# Autodesk Inventor assembly: GP6-100
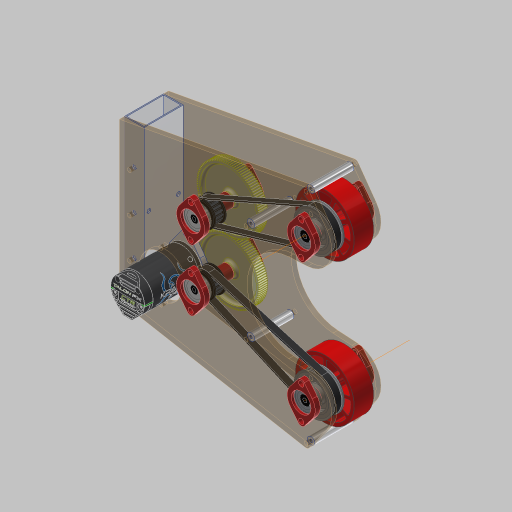
[picture p0: Inventor's stored thumbnail of the model, 512x512]
Saved by Autodesk Inventor 2023.5 (Build 275446000, 446)
## iProperties
Created: 2025-02-23
Part Number: GP6-100
Document SubType Name: Assembly
Designer: slick
Author: slick
## Documents named in this file (23)
- C:\Users\slick\OneDrive\Desktop\2025-ReefScape---CAD\Gripper\GP6\GP6-100.iam
- C:\Users\slick\OneDrive\Desktop\2025-ReefScape---CAD\Gripper\GP6\GP6-001.ipt
- C:\Users\slick\OneDrive\Desktop\2025-ReefScape---CAD\Gripper\GP6\GP6-003.ipt
- C:\Users\slick\OneDrive\Desktop\2025-ReefScape---CAD\Gripper\GP6\GP6-002.ipt
- C:\Users\slick\OneDrive\Desktop\2025-ReefScape---CAD\COMMON PARTS\BEARINGS\0_500_ID_x_1_125_OD_x_0_313_WD_Flanged_Bearing_217-2731.ipt
- C:\Users\slick\OneDrive\Desktop\2025-ReefScape---CAD\COMMON PARTS\BEARINGS\Bearing Retainer\Retainer.ipt
- C:\Users\slick\OneDrive\Desktop\2025-ReefScape---CAD\COMMON PARTS\BEARINGS\0_375_ID_x_1_125_OD_x_0_313_WD_Flanged_Bearing_217-2732.ipt
- C:\Users\slick\OneDrive\Desktop\2025-ReefScape---CAD\Gripper\GP6\GP6-005.ipt
- C:\Users\slick\OneDrive\Desktop\2025-ReefScape---CAD\Gripper\GP6\GP6-006.ipt
- C:\Users\slick\OneDrive\Desktop\2025-ReefScape---CAD\COMMON PARTS\GEARS\15t Spur Gear\15t Spur Gear.ipt
- C:\Users\slick\OneDrive\Desktop\2025-ReefScape---CAD\COMMON PARTS\GEARS\32 dp gear\100t_Aluminum_Spur_Gear_32_DP_3_8_Hex_Bore_217-5865.ipt
- C:\Users\slick\OneDrive\Desktop\2025-ReefScape---CAD\Gripper\GP6\GP6-007.ipt
- C:\Users\slick\OneDrive\Desktop\2025-ReefScape---CAD\COMMON PARTS\PULLEYS\htd\30t_x_9mm_Wide_Double_Flange_Aluminum_Pulley_HTD_5mm_1_2_Hex_Bore_217-3229.ipt
- C:\Users\slick\OneDrive\Desktop\2025-ReefScape---CAD\COMMON PARTS\PULLEYS\htd\18t_x_9mm_Wide_Double_Flange_Aluminum_Pulley_HTD_5mm_1_2_Hex_Bore_217-3225.ipt
- C:\Users\slick\OneDrive\Desktop\2025-ReefScape---CAD\COMMON PARTS\WHEELS\am-3946 3IN 375Hex Compliant Wheel REV 3.ipt
- C:\Users\slick\OneDrive\Desktop\2025-ReefScape---CAD\COMMON PARTS\MOTORS\WCP-0941 x44 Kracken.ipt
- C:\Users\slick\OneDrive\Desktop\2025-ReefScape---CAD\Gripper\GP6\GP6-008.ipt
- C:\Users\slick\OneDrive\Desktop\2025-ReefScape---CAD\Gripper\GP6\GP6-009.ipt
- C:\Users\slick\OneDrive\Desktop\2025-ReefScape---CAD\Gripper\GP6\GP6-010.ipt
- C:\Users\slick\OneDrive\Desktop\2025-ReefScape---CAD\Gripper\GP6\GP6-011.ipt
- C:\Users\slick\OneDrive\Desktop\2025-ReefScape---CAD\Gripper\GP6\GP6-012.ipt
- C:\Users\slick\OneDrive\Desktop\2025-ReefScape---CAD\Gripper\GP6\GP6-013.ipt
- C:\Users\slick\OneDrive\Desktop\2025-ReefScape---CAD\Gripper\GP6\GP6-014 - 85T belt.ipt
## Components (52 placed, 22 different names)
1. GP6-001:1 — Insert:1, Insert:2, Insert:35, Insert:36, Insert:41, Insert:42, Insert:43, Insert:46, Insert:47, Insert:54, Insert:55, Insert:60, Insert:61, Insert:62, Insert:63, Insert:65, Insert:66, Mate:25, Mate:27, Mate:42, Mate:43
2. GP6-003:1 — Insert:1, Insert:2, Insert:3, Insert:4
3. GP6-002:1 — Insert:3, Insert:4, Insert:38, Insert:39, Insert:40, Insert:44, Insert:45, Insert:48, Insert:49, Insert:50, Insert:51, Insert:52, Insert:53, Insert:56, Insert:57, Insert:58, Insert:59, Mate:29, Mate:31, Mate:33, Mate:34
4. GP6-005:1 — Insert:33, Insert:34, Mate:19, Insert:64
5. GP6-006:1 — Insert:33, Insert:35
6. GP6-006:2 — Insert:34, Insert:36
7. GP6-007:1 — Insert:38
8. GP6-007:2 — Insert:40
9. GP6-007:3 — Insert:41
10. GP6-007:4 — Insert:39
11. am-3946 3IN 375Hex Compliant Wheel REV 3:1 — Mate:9, Flush:5
12. am-3946 3IN 375Hex Compliant Wheel REV 3:4 — Mate:18, Flush:5, Mate:23, Mate:45
13. WCP-0941 x44 Kracken:1 — Mate:19, Insert:64, Mate:48, Mate:49
14. GP6-008:1 — Mate:20, Flush:6, Mate:35, Mate:37, Mate:41, Mate:44
15. GP6-008:2 — Flush:7, Mate:21, Mate:32, Mate:36, Mate:40, Mate:46
16. GP6-009:1 — Mate:23, Flush:9
17. GP6-009:2 — Mate:22, Flush:8
18. Retainer:8 — Insert:65, Insert:66
19. 0_375_ID_x_1_125_OD_x_0_313_WD_Flanged_Bearing_217-2732:4 — Insert:47
20. 0_375_ID_x_1_125_OD_x_0_313_WD_Flanged_Bearing_217-2732:3 — Insert:48, Mate:13, Mate:16, Mate:20, Flush:6
21. 0_375_ID_x_1_125_OD_x_0_313_WD_Flanged_Bearing_217-2732:2 — Insert:49, Mate:11
22. 0_375_ID_x_1_125_OD_x_0_313_WD_Flanged_Bearing_217-2732:1 — Insert:46, Mate:15, Flush:7, Mate:21
23. 0_500_ID_x_1_125_OD_x_0_313_WD_Flanged_Bearing_217-2731:4 — Insert:44, Mate:17, Mate:30
24. 0_500_ID_x_1_125_OD_x_0_313_WD_Flanged_Bearing_217-2731:3 — Insert:43, Flush:9, Mate:26
25. 0_500_ID_x_1_125_OD_x_0_313_WD_Flanged_Bearing_217-2731:2 — Insert:42, Mate:22, Flush:8, Mate:24, Mate:47
26. 0_500_ID_x_1_125_OD_x_0_313_WD_Flanged_Bearing_217-2731:1 — Insert:45, Mate:10, Mate:28
27. Retainer:7 — Insert:60, Insert:61
28. Retainer:6 — Insert:62, Insert:63
29. Retainer:5 — Insert:58, Insert:59
30. Retainer:4 — Insert:56, Insert:57
31. Retainer:3 — Insert:54, Insert:55
32. Retainer:2 — Insert:52, Insert:53
33. Retainer:1 — Insert:50, Insert:51
34. 100t_Aluminum_Spur_Gear_32_DP_3_8_Hex_Bore_217-5865:1 — Flush:1, Mate:12, Mate:15
35. 100t_Aluminum_Spur_Gear_32_DP_3_8_Hex_Bore_217-5865:2 — Flush:1, Mate:14
36. 30t_x_9mm_Wide_Double_Flange_Aluminum_Pulley_HTD_5mm_1_2_Hex_Bore_217-3229:1 — Flush:2, Flush:4, Mate:9, Mate:10
37. 30t_x_9mm_Wide_Double_Flange_Aluminum_Pulley_HTD_5mm_1_2_Hex_Bore_217-3229:2 — Flush:3, Flush:4, Mate:17, Mate:18
38. 18t_x_9mm_Wide_Double_Flange_Aluminum_Pulley_HTD_5mm_1_2_Hex_Bore_217-3225:1 — Flush:2, Mate:11, Mate:12, Mate:39, Flush:11
39. 18t_x_9mm_Wide_Double_Flange_Aluminum_Pulley_HTD_5mm_1_2_Hex_Bore_217-3225:2 — Flush:3, Mate:13, Mate:14, Mate:16, Mate:38, Flush:10
40. GP6-014 - 85T belt:1 — Mate:46, Mate:47, Flush:11
41. GP6-014 - 85T belt:2 — Mate:44, Mate:45, Flush:10
42. 15t Spur Gear:1 — Mate:48, Mate:49
43. GP6-010:1 — Mate:26, Mate:27
44. GP6-010:2 — Mate:24, Mate:25
45. GP6-011:1 — Mate:28, Mate:29
46. GP6-011:3 — Mate:30, Mate:31
47. GP6-012:1 — Mate:32, Mate:33
48. GP6-012:2 — Mate:34, Mate:35
49. GP6-013:1 — Mate:36, Mate:39
50. GP6-013:2 — Mate:37, Mate:38
51. GP6-012:3 — Mate:41, Mate:43
52. GP6-012:4 — Mate:40, Mate:42
## Relationships (89: Mate 41, Insert 37, Flush 11)
- Insert:1: GP6-001:1 ↔ GP6-003:1
- Insert:2: GP6-001:1 ↔ GP6-003:1
- Insert:3: GP6-003:1 ↔ GP6-002:1
- Insert:4: GP6-003:1 ↔ GP6-002:1
- Insert:33: GP6-005:1 ↔ GP6-006:1
- Insert:34: GP6-005:1 ↔ GP6-006:2
- Insert:35: GP6-001:1 ↔ GP6-006:1
- Insert:36: GP6-001:1 ↔ GP6-006:2
- Flush:1: 100t_Aluminum_Spur_Gear_32_DP_3_8_Hex_Bore_217-5865:1 ↔ 100t_Aluminum_Spur_Gear_32_DP_3_8_Hex_Bore_217-5865:2
- Insert:38: GP6-002:1 ↔ GP6-007:1
- Insert:39: GP6-002:1 ↔ GP6-007:4
- Insert:40: GP6-002:1 ↔ GP6-007:2
- Insert:41: GP6-001:1 ↔ GP6-007:3
- Flush:2: 30t_x_9mm_Wide_Double_Flange_Aluminum_Pulley_HTD_5mm_1_2_Hex_Bore_217-3229:1 ↔ 18t_x_9mm_Wide_Double_Flange_Aluminum_Pulley_HTD_5mm_1_2_Hex_Bore_217-3225:1
- Flush:3: 30t_x_9mm_Wide_Double_Flange_Aluminum_Pulley_HTD_5mm_1_2_Hex_Bore_217-3229:2 ↔ 18t_x_9mm_Wide_Double_Flange_Aluminum_Pulley_HTD_5mm_1_2_Hex_Bore_217-3225:2
- Flush:4: 30t_x_9mm_Wide_Double_Flange_Aluminum_Pulley_HTD_5mm_1_2_Hex_Bore_217-3229:1 ↔ 30t_x_9mm_Wide_Double_Flange_Aluminum_Pulley_HTD_5mm_1_2_Hex_Bore_217-3229:2
- Mate:9: am-3946 3IN 375Hex Compliant Wheel REV 3:1 ↔ 30t_x_9mm_Wide_Double_Flange_Aluminum_Pulley_HTD_5mm_1_2_Hex_Bore_217-3229:1
- Insert:42: GP6-001:1 ↔ 0_500_ID_x_1_125_OD_x_0_313_WD_Flanged_Bearing_217-2731:2
- Insert:43: GP6-001:1 ↔ 0_500_ID_x_1_125_OD_x_0_313_WD_Flanged_Bearing_217-2731:3
- Insert:44: GP6-002:1 ↔ 0_500_ID_x_1_125_OD_x_0_313_WD_Flanged_Bearing_217-2731:4
- Insert:45: GP6-002:1 ↔ 0_500_ID_x_1_125_OD_x_0_313_WD_Flanged_Bearing_217-2731:1
- Insert:46: GP6-001:1 ↔ 0_375_ID_x_1_125_OD_x_0_313_WD_Flanged_Bearing_217-2732:1
- Insert:47: GP6-001:1 ↔ 0_375_ID_x_1_125_OD_x_0_313_WD_Flanged_Bearing_217-2732:4
- Insert:48: GP6-002:1 ↔ 0_375_ID_x_1_125_OD_x_0_313_WD_Flanged_Bearing_217-2732:3
- Insert:49: GP6-002:1 ↔ 0_375_ID_x_1_125_OD_x_0_313_WD_Flanged_Bearing_217-2732:2
- Insert:50: GP6-002:1 ↔ Retainer:1
- Insert:51: GP6-002:1 ↔ Retainer:1
- Insert:52: GP6-002:1 ↔ Retainer:2
- Insert:53: GP6-002:1 ↔ Retainer:2
- Insert:54: GP6-001:1 ↔ Retainer:3
- Insert:55: GP6-001:1 ↔ Retainer:3
- Insert:56: GP6-002:1 ↔ Retainer:4
- Insert:57: GP6-002:1 ↔ Retainer:4
- Insert:58: GP6-002:1 ↔ Retainer:5
- Insert:59: GP6-002:1 ↔ Retainer:5
- Insert:60: GP6-001:1 ↔ Retainer:7
- Insert:61: GP6-001:1 ↔ Retainer:7
- Insert:62: GP6-001:1 ↔ Retainer:6
- Insert:63: GP6-001:1 ↔ Retainer:6
- Mate:10: 0_500_ID_x_1_125_OD_x_0_313_WD_Flanged_Bearing_217-2731:1 ↔ 30t_x_9mm_Wide_Double_Flange_Aluminum_Pulley_HTD_5mm_1_2_Hex_Bore_217-3229:1
- Mate:11: 0_375_ID_x_1_125_OD_x_0_313_WD_Flanged_Bearing_217-2732:2 ↔ 18t_x_9mm_Wide_Double_Flange_Aluminum_Pulley_HTD_5mm_1_2_Hex_Bore_217-3225:1
- Mate:12: 100t_Aluminum_Spur_Gear_32_DP_3_8_Hex_Bore_217-5865:1 ↔ 18t_x_9mm_Wide_Double_Flange_Aluminum_Pulley_HTD_5mm_1_2_Hex_Bore_217-3225:1
- Mate:13: 0_375_ID_x_1_125_OD_x_0_313_WD_Flanged_Bearing_217-2732:3 ↔ 18t_x_9mm_Wide_Double_Flange_Aluminum_Pulley_HTD_5mm_1_2_Hex_Bore_217-3225:2
- Mate:14: 100t_Aluminum_Spur_Gear_32_DP_3_8_Hex_Bore_217-5865:2 ↔ 18t_x_9mm_Wide_Double_Flange_Aluminum_Pulley_HTD_5mm_1_2_Hex_Bore_217-3225:2
- Mate:15 (3.175 mm): 0_375_ID_x_1_125_OD_x_0_313_WD_Flanged_Bearing_217-2732:1 ↔ 100t_Aluminum_Spur_Gear_32_DP_3_8_Hex_Bore_217-5865:1
- Mate:16 (3.175 mm): 0_375_ID_x_1_125_OD_x_0_313_WD_Flanged_Bearing_217-2732:3 ↔ 18t_x_9mm_Wide_Double_Flange_Aluminum_Pulley_HTD_5mm_1_2_Hex_Bore_217-3225:2
- Mate:17: 0_500_ID_x_1_125_OD_x_0_313_WD_Flanged_Bearing_217-2731:4 ↔ 30t_x_9mm_Wide_Double_Flange_Aluminum_Pulley_HTD_5mm_1_2_Hex_Bore_217-3229:2
- Mate:18: am-3946 3IN 375Hex Compliant Wheel REV 3:4 ↔ 30t_x_9mm_Wide_Double_Flange_Aluminum_Pulley_HTD_5mm_1_2_Hex_Bore_217-3229:2
- Flush:5: am-3946 3IN 375Hex Compliant Wheel REV 3:1 ↔ am-3946 3IN 375Hex Compliant Wheel REV 3:4
- Mate:19: GP6-005:1 ↔ WCP-0941 x44 Kracken:1
- Insert:64: GP6-005:1 ↔ WCP-0941 x44 Kracken:1
- Mate:20: GP6-008:1 ↔ 0_375_ID_x_1_125_OD_x_0_313_WD_Flanged_Bearing_217-2732:3
- Flush:6: GP6-008:1 ↔ 0_375_ID_x_1_125_OD_x_0_313_WD_Flanged_Bearing_217-2732:3
- Flush:7: GP6-008:2 ↔ 0_375_ID_x_1_125_OD_x_0_313_WD_Flanged_Bearing_217-2732:1
- Mate:21: GP6-008:2 ↔ 0_375_ID_x_1_125_OD_x_0_313_WD_Flanged_Bearing_217-2732:1
- Mate:22: GP6-009:2 ↔ 0_500_ID_x_1_125_OD_x_0_313_WD_Flanged_Bearing_217-2731:2
- Mate:23: am-3946 3IN 375Hex Compliant Wheel REV 3:4 ↔ GP6-009:1
- Flush:8: GP6-009:2 ↔ 0_500_ID_x_1_125_OD_x_0_313_WD_Flanged_Bearing_217-2731:2
- Flush:9: GP6-009:1 ↔ 0_500_ID_x_1_125_OD_x_0_313_WD_Flanged_Bearing_217-2731:3
- Insert:65: GP6-001:1 ↔ Retainer:8
- Insert:66: GP6-001:1 ↔ Retainer:8
- Mate:24: 0_500_ID_x_1_125_OD_x_0_313_WD_Flanged_Bearing_217-2731:2 ↔ GP6-010:2
- Mate:25: GP6-001:1 ↔ GP6-010:2
- Mate:26: 0_500_ID_x_1_125_OD_x_0_313_WD_Flanged_Bearing_217-2731:3 ↔ GP6-010:1
- Mate:27: GP6-001:1 ↔ GP6-010:1
- Mate:28: 0_500_ID_x_1_125_OD_x_0_313_WD_Flanged_Bearing_217-2731:1 ↔ GP6-011:1
- Mate:29: GP6-002:1 ↔ GP6-011:1
- Mate:30: 0_500_ID_x_1_125_OD_x_0_313_WD_Flanged_Bearing_217-2731:4 ↔ GP6-011:3
- Mate:31: GP6-002:1 ↔ GP6-011:3
- Mate:32: GP6-008:2 ↔ GP6-012:1
- Mate:33: GP6-002:1 ↔ GP6-012:1
- Mate:34: GP6-002:1 ↔ GP6-012:2
- Mate:35: GP6-008:1 ↔ GP6-012:2
- Mate:36: GP6-008:2 ↔ GP6-013:1
- Mate:37: GP6-008:1 ↔ GP6-013:2
- Mate:38: 18t_x_9mm_Wide_Double_Flange_Aluminum_Pulley_HTD_5mm_1_2_Hex_Bore_217-3225:2 ↔ GP6-013:2
- Mate:39: 18t_x_9mm_Wide_Double_Flange_Aluminum_Pulley_HTD_5mm_1_2_Hex_Bore_217-3225:1 ↔ GP6-013:1
- Mate:40: GP6-008:2 ↔ GP6-012:4
- Mate:41: GP6-008:1 ↔ GP6-012:3
- Mate:42: GP6-001:1 ↔ GP6-012:4
- Mate:43: GP6-001:1 ↔ GP6-012:3
- Mate:44: GP6-008:1 ↔ GP6-014 - 85T belt:2
- Mate:45 (0.0762 mm): am-3946 3IN 375Hex Compliant Wheel REV 3:4 ↔ GP6-014 - 85T belt:2
- Mate:46: GP6-008:2 ↔ GP6-014 - 85T belt:1
- Mate:47 (0.0762 mm): 0_500_ID_x_1_125_OD_x_0_313_WD_Flanged_Bearing_217-2731:2 ↔ GP6-014 - 85T belt:1
- Flush:10: 18t_x_9mm_Wide_Double_Flange_Aluminum_Pulley_HTD_5mm_1_2_Hex_Bore_217-3225:2 ↔ GP6-014 - 85T belt:2
- Flush:11: 18t_x_9mm_Wide_Double_Flange_Aluminum_Pulley_HTD_5mm_1_2_Hex_Bore_217-3225:1 ↔ GP6-014 - 85T belt:1
- Mate:48: WCP-0941 x44 Kracken:1 ↔ 15t Spur Gear:1
- Mate:49: WCP-0941 x44 Kracken:1 ↔ 15t Spur Gear:1
